# Autodesk Inventor assembly: Micromouse 2019 (14HM08)
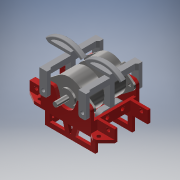
[picture p0: Inventor's stored thumbnail of the model, 180x180]
Saved by Autodesk Inventor 2019 (Build 230136000, 136)
## iProperties
Created: 2019-02-17
Part Number: Micromouse 2019 (14HM08)
Document SubType Name: Assembly
Designer: Billy
Author: Billy
## Documents named in this file (7)
- C:\Users\billy_000\Documents\Micromouse\2019\Design Files\CAD\Micromouse 2019 (14HM08).iam
- C:\Users\billy_000\Documents\Micromouse\2019\Design Files\CAD\14HM08 Chassis.ipt
- C:\Users\billy_000\Documents\Micromouse\2019\Design Files\CAD\14HM08.ipt
- C:\Users\billy_000\Documents\Micromouse\2019\Design Files\CAD\14HM08 Chassis Sleds.ipt
- C:\Users\billy_000\Documents\Micromouse\2019\SensorBoard\Sensor Board.ipt
- C:\Users\billy_000\Documents\Micromouse\2019\Design Files\CAD\pololu-wheel-60×8mm\pololu-wheel-60x8mm-black.ipt
- C:\Users\billy_000\Documents\Micromouse\2019\Design Files\CAD\pololu-universal-aluminum-mounting-hub-for-5mm-shaft-4-40-holes.ipt
## Components (15 placed, 6 different names)
1. 14HM08 Chassis:1 — Insert:1, Insert:2, Insert:3, Insert:4, Insert:7, Insert:8, Insert:9, Insert:10, Angle:1, Angle:2, Insert:11, Insert:12, Insert:13, Insert:14, Angle:3, Angle:4, Angle:5, Angle:6, Insert:21, Insert:22
2. 14HM08:1 — Insert:1, Insert:2, Insert:19
3. 14HM08:2 — Insert:3, Insert:4, Insert:20
4. 14HM08 Chassis Sleds:1 — Insert:7, Insert:8
5. Sensor Board:1 — Insert:9, Angle:2
6. Sensor Board:2 — Insert:10, Angle:1
7. Sensor Board:3 — Insert:11, Angle:4
8. Sensor Board:4 — Insert:12, Angle:5
9. Sensor Board:5 — Insert:13, Angle:6
10. Sensor Board:6 — Insert:14, Angle:3
11. pololu-wheel-60x8mm-black:1 — Insert:17, Insert:18
12. pololu-wheel-60x8mm-black:2 — Insert:15, Insert:16
13. pololu-universal-aluminum-mounting-hub-for-5mm-shaft-4-40-holes:1 — Insert:15, Insert:16, Insert:19
14. pololu-universal-aluminum-mounting-hub-for-5mm-shaft-4-40-holes:2 — Insert:17, Insert:18, Insert:20
15. 14HM08 Chassis Sleds:2 — Insert:21, Insert:22
## Relationships (26: Insert 20, Angle 6)
- Insert:1: 14HM08 Chassis:1 ↔ 14HM08:1
- Insert:2: 14HM08 Chassis:1 ↔ 14HM08:1
- Insert:3: 14HM08 Chassis:1 ↔ 14HM08:2
- Insert:4: 14HM08 Chassis:1 ↔ 14HM08:2
- Insert:7: 14HM08 Chassis:1 ↔ 14HM08 Chassis Sleds:1
- Insert:8: 14HM08 Chassis:1 ↔ 14HM08 Chassis Sleds:1
- Insert:9: 14HM08 Chassis:1 ↔ Sensor Board:1
- Insert:10: 14HM08 Chassis:1 ↔ Sensor Board:2
- Angle:1 (180 deg): 14HM08 Chassis:1 ↔ Sensor Board:2
- Angle:2 (180 deg): 14HM08 Chassis:1 ↔ Sensor Board:1
- Insert:11: 14HM08 Chassis:1 ↔ Sensor Board:3
- Insert:12: 14HM08 Chassis:1 ↔ Sensor Board:4
- Insert:13: 14HM08 Chassis:1 ↔ Sensor Board:5
- Insert:14: 14HM08 Chassis:1 ↔ Sensor Board:6
- Angle:3 (180 deg): 14HM08 Chassis:1 ↔ Sensor Board:6
- Angle:4 (180 deg): 14HM08 Chassis:1 ↔ Sensor Board:3
- Angle:5 (180 deg): 14HM08 Chassis:1 ↔ Sensor Board:4
- Angle:6 (180 deg): 14HM08 Chassis:1 ↔ Sensor Board:5
- Insert:15: pololu-wheel-60x8mm-black:2 ↔ pololu-universal-aluminum-mounting-hub-for-5mm-shaft-4-40-holes:1
- Insert:16: pololu-wheel-60x8mm-black:2 ↔ pololu-universal-aluminum-mounting-hub-for-5mm-shaft-4-40-holes:1
- Insert:17: pololu-wheel-60x8mm-black:1 ↔ pololu-universal-aluminum-mounting-hub-for-5mm-shaft-4-40-holes:2
- Insert:18: pololu-wheel-60x8mm-black:1 ↔ pololu-universal-aluminum-mounting-hub-for-5mm-shaft-4-40-holes:2
- Insert:19 (-12 mm): 14HM08:1 ↔ pololu-universal-aluminum-mounting-hub-for-5mm-shaft-4-40-holes:1
- Insert:20 (-12 mm): 14HM08:2 ↔ pololu-universal-aluminum-mounting-hub-for-5mm-shaft-4-40-holes:2
- Insert:21: 14HM08 Chassis:1 ↔ 14HM08 Chassis Sleds:2
- Insert:22: 14HM08 Chassis:1 ↔ 14HM08 Chassis Sleds:2
